# Autodesk Inventor assembly: сервоприводы
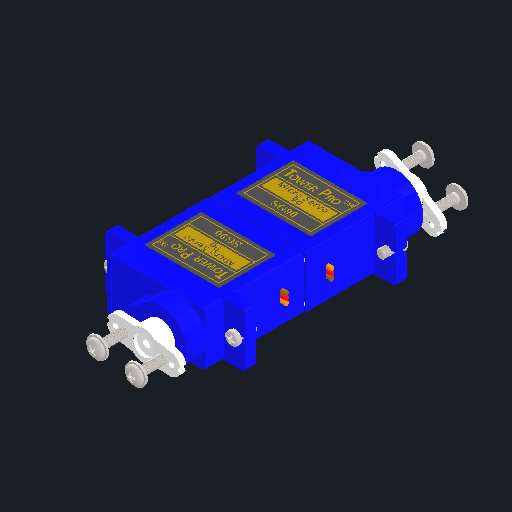
[picture p0: Inventor's stored thumbnail of the model, 512x512]
Saved by Autodesk Inventor 2022 (Build 260153000, 153)
## iProperties
Created: 2025-02-01
Part Number: сервоприводы
Document SubType Name: Assembly
Designer: it
Author: it
## Documents named in this file (4)
- E:\машина\сервоприводы.iam
- E:\машина\сервы2.iam
- E:\abuyz lkz vfibyrb\SG90 - Micro Servo 9g - Tower Pro.5_BS EN ISO 7045 - M2 x 8 - Z - 8S.ipt
- E:\машина\сервы.iam
## Components (6 placed, 3 different names)
1. сервы2:1 [sub-assembly]
2. SG90 - Micro Servo 9g - Tower Pro.5_BS EN ISO 7045 - M2 x 8 - Z - 8S:1
3. SG90 - Micro Servo 9g - Tower Pro.5_BS EN ISO 7045 - M2 x 8 - Z - 8S:2
4. SG90 - Micro Servo 9g - Tower Pro.5_BS EN ISO 7045 - M2 x 8 - Z - 8S:3
5. SG90 - Micro Servo 9g - Tower Pro.5_BS EN ISO 7045 - M2 x 8 - Z - 8S:4
6. сервы:1 [sub-assembly]
## Relationships (4: Mate 4)
- [Mate]: сервы2:1 ↔ сервы:1
- [Mate]: сервы2:1 ↔ сервы:1
- [Mate]: сервы2:1 ↔ сервы:1
- [Mate]: сервы2:1 ↔ сервы:1
